# Autodesk Inventor assembly: Link_03_Assembly_V02
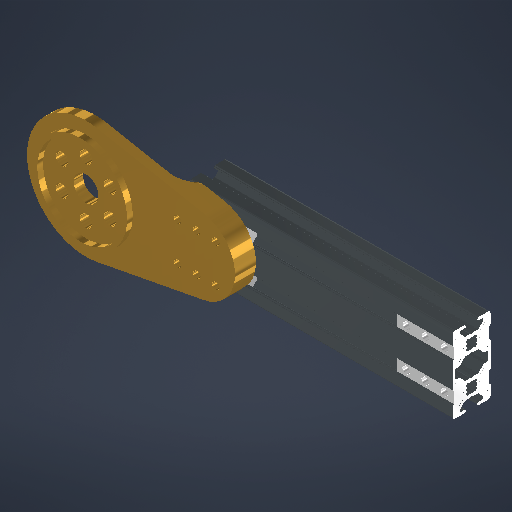
[picture p0: Inventor's stored thumbnail of the model, 512x512]
Saved by Autodesk Inventor 2026 (Build 300175000, 175)
## iProperties
Created: 2025-12-01
Part Number: Link_03_Assembly_V02
Document SubType Name: Assembly
Designer: DanielFGarzon
Mass: 165.359 g
Surface Area: 681.236 cm^2
Volume: 81.4726 cm^3
Density: 2.02963 g/cm^3
Author: DanielFGarzon
## Documents named in this file (3)
- D:\POLIMI\3RD SEMESTER\Industrial Robotics\Project\Mine\Inventor_Files\Link_03_Assembly_V04.iam
- D:\POLIMI\3RD SEMESTER\Industrial Robotics\Project\Mine\Inventor_Files\Link_03_V03.ipt
- D:\POLIMI\3RD SEMESTER\Industrial Robotics\Project\Mine\Inventor_Files\Reducer_02\RotationalConector_20x40.ipt
## Components (2 placed, 2 different names)
1. Link_03_V03:1 — Flush:1, Flush:2, Mate:2, Mate:3, Mate:4
2. RotationalConector_20x40:1 — Mate:1, Mate:2, Mate:3, Mate:4
## Relationships (6: Mate 4, Flush 2)
- Flush:1: Link_03_V03:1
- Flush:2: Link_03_V03:1
- Mate:1: RotationalConector_20x40:1
- Mate:2: Link_03_V03:1 ↔ RotationalConector_20x40:1
- Mate:3: Link_03_V03:1 ↔ RotationalConector_20x40:1
- Mate:4: Link_03_V03:1 ↔ RotationalConector_20x40:1
